# Autodesk Inventor assembly: Krystal
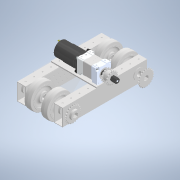
[picture p0: Inventor's stored thumbnail of the model, 180x180]
Saved by Autodesk Inventor 2020 (Build 240168000, 168)
## iProperties
Created: 2020-02-03
Part Number: Krystal
Document SubType Name: Assembly
Designer: aidan
Author: aidan
## Documents named in this file (9)
- C:\Users\aidan\Desktop\T3 Robotics\CAD\Krystal.iam
- C:\Users\aidan\Desktop\T3 Robotics\CAD\VerseFrame 10in KY.ipt
- C:\Users\aidan\Desktop\T3 Robotics\CAD\Generic and Stock\Colson 3x.875.ipt
- C:\Users\aidan\Desktop\T3 Robotics\CAD\Generic and Stock\double bearing.iam
- C:\Users\aidan\Desktop\T3 Robotics\CAD\Generic and Stock\22T 22 Sprocket.ipt
- C:\Users\aidan\Desktop\T3 Robotics\CAD\Flat Bar KY.ipt
- C:\Users\aidan\Desktop\T3 Robotics\CAD\Generic and Stock\VersaPlanetary Parts\VersaPlanetary Two Stage 775.iam
- C:\Users\aidan\Desktop\T3 Robotics\CAD\Generic and Stock\16T 22 Sprocket.ipt
- C:\Users\aidan\Desktop\T3 Robotics\CAD\Krystal Plate.ipt
## Components (18 placed, 8 different names)
1. VerseFrame 10in KY:1 — Flush:1, Flush:2, Mate:1, Mate:4, Mate:6, Flush:14, Mate:26, Flush:15, Mate:27
2. VerseFrame 10in KY:2 — Flush:1, Flush:2, Mate:2, Mate:3, Mate:5, Mate:16, Flush:11, Mate:17
3. Colson 3x.875:1 — Flush:3, Flush:6, Mate:9, Flush:10, Mate:10
4. Colson 3x.875:2 — Flush:4, Flush:5, Flush:9
5. Colson 3x.875:3 — Flush:3, Flush:6, Mate:7, Mate:9, Flush:9, Mate:11
6. Colson 3x.875:4 — Flush:4, Flush:5, Mate:8, Flush:10
7. double bearing:1 [sub-assembly] — Mate:1, Flush:7, Mate:6, Mate:7, Mate:10
8. double bearing:2 [sub-assembly] — Mate:4, Flush:7, Mate:8
9. double bearing:3 [sub-assembly] — Mate:2, Flush:8, Mate:5, Mate:11, Mate:13, Mate:15
10. double bearing:4 [sub-assembly] — Mate:3, Flush:8, Mate:14
11. 22T 22 Sprocket:1 — Mate:12, Mate:13, Mate:15
12. 22T 22 Sprocket:2 — Mate:12, Mate:14, Flush:13
13. Flat Bar KY:1 — Mate:16, Flush:11, Mate:17, Mate:18, Mate:19, Mate:20, Mate:21
14. VersaPlanetary Two Stage 775:1 [sub-assembly] — Mate:18, Mate:19, Mate:20, Mate:21, Mate:23, Mate:25
15. 16T 22 Sprocket:1 — Flush:12, Mate:22, Mate:24, Flush:13, Mate:25
16. 16T 22 Sprocket:2 — Flush:12, Mate:22, Mate:23, Mate:24
17. Krystal Plate:1 — Flush:14, Mate:26, Flush:15, Mate:28, Flush:16
18. Krystal Plate:2 — Mate:27, Mate:28, Flush:16
## Relationships (44: Mate 28, Flush 16)
- Flush:1: VerseFrame 10in KY:1 ↔ VerseFrame 10in KY:2
- Flush:2: VerseFrame 10in KY:1 ↔ VerseFrame 10in KY:2
- Flush:3: Colson 3x.875:1 ↔ Colson 3x.875:3
- Flush:4: Colson 3x.875:2 ↔ Colson 3x.875:4
- Flush:5: Colson 3x.875:2 ↔ Colson 3x.875:4
- Flush:6: Colson 3x.875:1 ↔ Colson 3x.875:3
- Mate:1: VerseFrame 10in KY:1 ↔ double bearing:1
- Mate:2: VerseFrame 10in KY:2 ↔ double bearing:3
- Mate:3: VerseFrame 10in KY:2 ↔ double bearing:4
- Mate:4: VerseFrame 10in KY:1 ↔ double bearing:2
- Flush:7: double bearing:1 ↔ double bearing:2
- Flush:8: double bearing:3 ↔ double bearing:4
- Mate:5: VerseFrame 10in KY:2 ↔ double bearing:3
- Mate:6: VerseFrame 10in KY:1 ↔ double bearing:1
- Mate:7: Colson 3x.875:3 ↔ double bearing:1
- Mate:8: Colson 3x.875:4 ↔ double bearing:2
- Mate:9 (22.225 mm): Colson 3x.875:1 ↔ Colson 3x.875:3
- Flush:9: Colson 3x.875:2 ↔ Colson 3x.875:3
- Flush:10: Colson 3x.875:1 ↔ Colson 3x.875:4
- Mate:10 (3.175 mm): Colson 3x.875:1 ↔ double bearing:1
- Mate:11 (3.175 mm): Colson 3x.875:3 ↔ double bearing:3
- Mate:12: 22T 22 Sprocket:1 ↔ 22T 22 Sprocket:2
- Mate:13: double bearing:3 ↔ 22T 22 Sprocket:1
- Mate:14: double bearing:4 ↔ 22T 22 Sprocket:2
- Mate:15 (3.175 mm): double bearing:3 ↔ 22T 22 Sprocket:1
- Mate:16: VerseFrame 10in KY:2 ↔ Flat Bar KY:1
- Flush:11: VerseFrame 10in KY:2 ↔ Flat Bar KY:1
- Mate:17: VerseFrame 10in KY:2 ↔ Flat Bar KY:1
- Mate:18: Flat Bar KY:1 ↔ VersaPlanetary Two Stage 775:1
- Mate:19: Flat Bar KY:1 ↔ VersaPlanetary Two Stage 775:1
- Mate:20: Flat Bar KY:1 ↔ VersaPlanetary Two Stage 775:1
- Mate:21: Flat Bar KY:1 ↔ VersaPlanetary Two Stage 775:1
- Flush:12: 16T 22 Sprocket:1 ↔ 16T 22 Sprocket:2
- Mate:22: 16T 22 Sprocket:1 ↔ 16T 22 Sprocket:2
- Mate:23: VersaPlanetary Two Stage 775:1 ↔ 16T 22 Sprocket:2
- Mate:24: 16T 22 Sprocket:1 ↔ 16T 22 Sprocket:2
- Flush:13: 22T 22 Sprocket:2 ↔ 16T 22 Sprocket:1
- Mate:25: VersaPlanetary Two Stage 775:1 ↔ 16T 22 Sprocket:1
- Flush:14: VerseFrame 10in KY:1 ↔ Krystal Plate:1
- Mate:26: VerseFrame 10in KY:1 ↔ Krystal Plate:1
- Flush:15 (-50.8 mm): VerseFrame 10in KY:1 ↔ Krystal Plate:1
- Mate:27: VerseFrame 10in KY:1 ↔ Krystal Plate:2
- Mate:28: Krystal Plate:1 ↔ Krystal Plate:2
- Flush:16: Krystal Plate:1 ↔ Krystal Plate:2
